# Autodesk Inventor assembly: BatteryRackk-Assembly
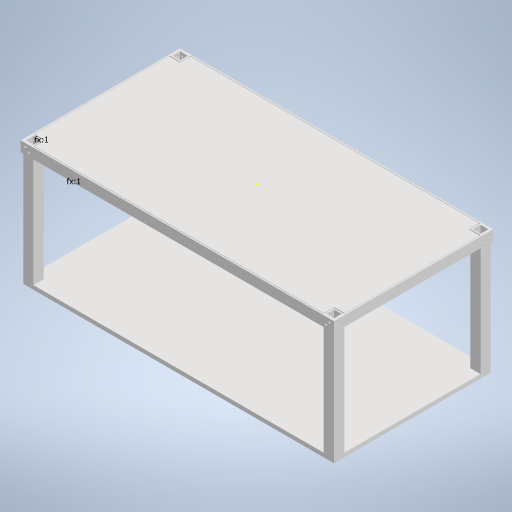
[picture p0: Inventor's stored thumbnail of the model, 512x512]
Saved by Autodesk Inventor 2023 (Build 270158000, 158)
## iProperties
Created: 2023-06-24
Part Number: BatteryRackk-Assembly
Document SubType Name: Assembly
Designer: incep
Author: incep
## Documents named in this file (6)
- C:\Projects\TechnoGecko\TechnoGecko-BatteryRack\BatteryRackk-Assembly.iam
- C:\Projects\TechnoGecko\TechnoGecko-BatteryRack\assyBase.ipt
- C:\Projects\TechnoGecko\TechnoGecko-BatteryRack\vertical.ipt
- C:\Projects\TechnoGecko\TechnoGecko-BatteryRack\beamX.ipt
- C:\Projects\TechnoGecko\TechnoGecko-BatteryRack\beamZ.ipt
- C:\Projects\TechnoGecko\TechnoGecko-BatteryRack\shelf.ipt
## Components (10 placed, 5 different names)
1. assyBase:1 — Mate:1, Mate:2, Mate:3, Mate:4, Flush:1, Flush:2, Mate:5, Mate:6, Flush:3, Flush:4, Mate:7, Flush:5, Flush:6, Mate:8, Flush:7, Flush:8
2. vertical:1 — Flush:1, Flush:2, Mate:5, Flush:10, Mate:12, Flush:11
3. vertical:2 — Mate:6, Flush:3, Flush:4, Flush:9, Mate:9, Mate:10, Mate:11, Mate:15, Mate:16, Mate:17
4. vertical:3 — Mate:7, Flush:5, Flush:6, Mate:19, Mate:20
5. vertical:4 — Mate:8, Flush:7, Flush:8, Mate:13, Mate:14, Flush:12, Mate:18
6. beamX:1 — Flush:9, Mate:9, Mate:10, Mate:11
7. beamX:2 — Flush:10, Mate:12, Mate:13, Mate:14, Mate:23
8. beamZ:1 — Flush:11, Mate:15, Mate:16, Mate:17, Mate:21
9. beamZ:2 — Flush:12, Mate:18, Mate:19, Mate:20, Mate:22
10. shelf:1 — Mate:21, Mate:22, Mate:23
## Relationships (35: Mate 23, Flush 12)
- Mate:1: assyBase:1
- Mate:2: assyBase:1
- Mate:3: assyBase:1
- Mate:4: assyBase:1
- Flush:1: assyBase:1 ↔ vertical:1
- Flush:2: assyBase:1 ↔ vertical:1
- Mate:5: assyBase:1 ↔ vertical:1
- Mate:6: assyBase:1 ↔ vertical:2
- Flush:3: assyBase:1 ↔ vertical:2
- Flush:4: assyBase:1 ↔ vertical:2
- Mate:7: assyBase:1 ↔ vertical:3
- Flush:5: assyBase:1 ↔ vertical:3
- Flush:6: assyBase:1 ↔ vertical:3
- Mate:8: assyBase:1 ↔ vertical:4
- Flush:7: assyBase:1 ↔ vertical:4
- Flush:8: assyBase:1 ↔ vertical:4
- Flush:9: vertical:2 ↔ beamX:1
- Mate:9: vertical:2 ↔ beamX:1
- Mate:10: vertical:2 ↔ beamX:1
- Mate:11: vertical:2 ↔ beamX:1
- Flush:10: vertical:1 ↔ beamX:2
- Mate:12: vertical:1 ↔ beamX:2
- Mate:13: vertical:4 ↔ beamX:2
- Mate:14: vertical:4 ↔ beamX:2
- Flush:11: vertical:1 ↔ beamZ:1
- Mate:15: vertical:2 ↔ beamZ:1
- Mate:16: vertical:2 ↔ beamZ:1
- Mate:17: vertical:2 ↔ beamZ:1
- Flush:12: vertical:4 ↔ beamZ:2
- Mate:18: vertical:4 ↔ beamZ:2
- Mate:19: vertical:3 ↔ beamZ:2
- Mate:20: vertical:3 ↔ beamZ:2
- Mate:21: beamZ:1 ↔ shelf:1
- Mate:22 (1 mm): beamZ:2 ↔ shelf:1
- Mate:23 (1 mm): beamX:2 ↔ shelf:1
